# Autodesk Inventor assembly: Link2
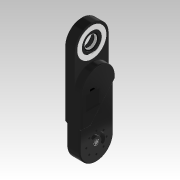
[picture p0: Inventor's stored thumbnail of the model, 180x180]
Saved by Autodesk Inventor 2020 (Build 240168000, 168)
## iProperties
Created: 2021-11-29
Part Number: Link2
Document SubType Name: Assembly
Designer: DDeGo
Author: DDeGo
## Documents named in this file (10)
- C:\Users\DDeGo\Documents\Drew\Projects\OS-ARM\cad\FirstDraft\Link2.iam
- C:\Users\DDeGo\Documents\Drew\Projects\OS-ARM\cad\FirstDraft\Link2a.ipt
- C:\Users\DDeGo\Documents\Drew\Projects\OS-ARM\cad\FirstDraft\Link2b.ipt
- C:\Users\DDeGo\Documents\Drew\Projects\OS-ARM\cad\OTS\Other\CF Tube 4x2x100.ipt
- C:\Users\DDeGo\Documents\Drew\Projects\OS-ARM\cad\OTS\Other\CF Tube 6x4x200.ipt
- C:\Users\DDeGo\Documents\Drew\Projects\OS-ARM\cad\OTS\Electronics\Nema 17 22mm.ipt
- C:\Users\DDeGo\Documents\Drew\Projects\OS-ARM\cad\OTS\Thrust Bearings\AXK6085 thrust bearing.ipt
- C:\Users\DDeGo\Documents\Drew\Projects\OS-ARM\cad\OTS\Radial Bearings\6807 bearing.ipt
- C:\Users\DDeGo\Documents\Drew\Projects\OS-ARM\cad\OTS\Radial Bearings\688 bearing.ipt
- C:\Users\DDeGo\Documents\Drew\Projects\OS-ARM\cad\OTS\Other\GT2 20T Drive Pulley.ipt
## Components (12 placed, 9 different names)
1. Link2a:1 — Mate:1, Mate:2, Mate:3, Mate:4, Mate:5, Mate:6, Mate:9, Mate:17, Mate:18, Mate:19, Mate:20
2. Link2b:1 — Mate:7, Mate:8, Mate:9, Mate:10, Mate:11, Mate:12, Mate:13, Mate:14, Mate:15, Mate:16
3. CF Tube 4x2x100:1 — Mate:4, Flush:2
4. CF Tube 6x4x200:1 — Mate:2, Flush:1, Mate:5, Mate:7
5. CF Tube 6x4x200:2 — Mate:1, Flush:1, Mate:8
6. CF Tube 4x2x100:2 — Mate:3, Flush:2, Mate:6
7. Nema 17 22mm:1 — Mate:10, Mate:11, Mate:12, Mate:21
8. AXK6085 thrust bearing:1 — Mate:13, Mate:14
9. 6807 bearing:1 — Mate:15, Mate:16
10. 688 bearing:1 — Mate:17, Mate:20
11. 688 bearing:2 — Mate:18, Mate:19
12. GT2 20T Drive Pulley:1 — Mate:21
## Relationships (23: Mate 21, Flush 2)
- Mate:1: Link2a:1 ↔ CF Tube 6x4x200:2
- Mate:2: Link2a:1 ↔ CF Tube 6x4x200:1
- Mate:3: Link2a:1 ↔ CF Tube 4x2x100:2
- Mate:4: Link2a:1 ↔ CF Tube 4x2x100:1
- Flush:1: CF Tube 6x4x200:1 ↔ CF Tube 6x4x200:2
- Flush:2: CF Tube 4x2x100:1 ↔ CF Tube 4x2x100:2
- Mate:5: Link2a:1 ↔ CF Tube 6x4x200:1
- Mate:6: Link2a:1 ↔ CF Tube 4x2x100:2
- Mate:7: Link2b:1 ↔ CF Tube 6x4x200:1
- Mate:8: Link2b:1 ↔ CF Tube 6x4x200:2
- Mate:9: Link2a:1 ↔ Link2b:1
- Mate:10: Link2b:1 ↔ Nema 17 22mm:1
- Mate:11: Link2b:1 ↔ Nema 17 22mm:1
- Mate:12: Link2b:1 ↔ Nema 17 22mm:1
- Mate:13: Link2b:1 ↔ AXK6085 thrust bearing:1
- Mate:14: Link2b:1 ↔ AXK6085 thrust bearing:1
- Mate:15: Link2b:1 ↔ 6807 bearing:1
- Mate:16: Link2b:1 ↔ 6807 bearing:1
- Mate:17: Link2a:1 ↔ 688 bearing:1
- Mate:18: Link2a:1 ↔ 688 bearing:2
- Mate:19: Link2a:1 ↔ 688 bearing:2
- Mate:20: Link2a:1 ↔ 688 bearing:1
- Mate:21: Nema 17 22mm:1 ↔ GT2 20T Drive Pulley:1
